# Autodesk Inventor assembly: Ensamblaje
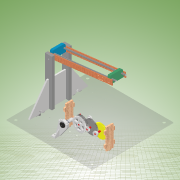
[picture p0: Inventor's stored thumbnail of the model, 180x180]
Saved by Autodesk Inventor 2022 (Build 260153000, 153)
## iProperties
Created: 2022-02-04
Part Number: Ensamblaje
Document SubType Name: Assembly
Designer: Marco
Author: Marco
## Documents named in this file (23)
- C:\Users\steff\Desktop\9noSemestre\Diseño\MiniProyecto\Ensamblaje.iam
- C:\Users\steff\Desktop\9noSemestre\Diseño\MiniProyecto\SoporteDerecha.ipt
- C:\Users\steff\Desktop\9noSemestre\Diseño\MiniProyecto\Varilla.ipt
- C:\Users\steff\Desktop\9noSemestre\Diseño\MiniProyecto\Riel_Lateral_MDF.ipt
- C:\Users\steff\Desktop\9noSemestre\Diseño\MiniProyecto\ColumnaSoporte.ipt
- C:\Users\steff\Desktop\9noSemestre\Diseño\MiniProyecto\SoporteIzquierda.ipt
- C:\Users\steff\Desktop\9noSemestre\Diseño\MiniProyecto\UnionColumnas.ipt
- C:\Users\steff\Desktop\9noSemestre\Diseño\MiniProyecto\SoporteMotor.ipt
- C:\Users\steff\Desktop\9noSemestre\Diseño\MiniProyecto\BaseProyecto.ipt
- C:\Users\steff\Desktop\9noSemestre\Diseño\MiniProyecto\SoporteMotorCierre.ipt
- C:\Users\steff\Desktop\9noSemestre\Diseño\MiniProyecto\dc motor.ipt
- C:\Users\steff\Desktop\9noSemestre\Diseño\MiniProyecto\CaraLateral.ipt
- C:\Users\steff\Desktop\9noSemestre\Diseño\MiniProyecto\Caja_CaraFrontal.ipt
- C:\Users\steff\Desktop\9noSemestre\Diseño\MiniProyecto\AcopleMotor.ipt
- C:\Users\steff\Desktop\9noSemestre\Diseño\MiniProyecto\SoporteEje.ipt
- C:\Users\steff\Desktop\9noSemestre\Diseño\MiniProyecto\Eje.ipt
- C:\Users\steff\Desktop\9noSemestre\Diseño\MiniProyecto\Engranaje.ipt
- C:\Users\steff\Desktop\9noSemestre\Diseño\MiniProyecto\EnsamblajesJuntos.iam
- C:\Users\steff\Desktop\9noSemestre\Diseño\MiniProyecto\libreria\es-ES\AS 1110\AS 1110 - M5 x 16.ipt
- C:\Users\steff\Desktop\9noSemestre\Diseño\MiniProyecto\Transmision_Inf.ipt
- C:\Users\steff\Desktop\9noSemestre\Diseño\MiniProyecto\Transmision_Sup.ipt
- C:\Users\steff\Desktop\9noSemestre\Diseño\MiniProyecto\Engranaje1.ipt
- C:\Users\steff\Desktop\9noSemestre\Diseño\MiniProyecto\Piñon1.ipt
## Components (36 placed, 22 different names)
1. ColumnaSoporte:1 — Coincidencia:1, Coincidencia:3, Coincidencia:6, Coincidencia:8, De rotación:2
2. ColumnaSoporte:2 — Coincidencia:2, Coincidencia:4, Coincidencia:5, Coincidencia:7, De rotación:1
3. UnionColumnas:1 — Coincidencia:3, Coincidencia:4, Coincidencia:5, Coincidencia:6, Coincidencia:21, Coincidencia:31, Coincidencia:92, Coincidencia:93
4. Riel_Lateral_MDF:1 — Coincidencia:7, De rotación:1, Coincidencia:10, Coincidencia:13, Coincidencia:14
5. Riel_Lateral_MDF:2 — Coincidencia:8, De rotación:2, De rotación:3, Coincidencia:9, Coincidencia:11, Coincidencia:12, Coincidencia:90
6. SoporteIzquierda:1 — De rotación:3, Coincidencia:9, Coincidencia:10, Coincidencia:15, Coincidencia:17, Coincidencia:18, Coincidencia:20
7. SoporteDerecha:1 — Coincidencia:11, Coincidencia:12, Coincidencia:13, Coincidencia:14, Coincidencia:16, Coincidencia:19
8. Varilla:1 — Coincidencia:15, Coincidencia:16, Coincidencia:17
9. Varilla:2 — Coincidencia:18, Coincidencia:19, Coincidencia:20
10. AS 1110 - Métrico M5 x 16:1 — Coincidencia:21
11. BaseProyecto:1 — Coincidencia:31, Coincidencia:46, Coincidencia:47, Coincidencia:92, Coincidencia:93, Coincidencia:94, Coincidencia:95
12. SoporteMotor:1 — Coincidencia:32, Coincidencia:33, Coincidencia:34, Coincidencia:35, Coincidencia:47, Coincidencia:48, Coincidencia:49
13. SoporteMotorCierre:1 — Coincidencia:32, Coincidencia:33, Coincidencia:34, Coincidencia:50
14. dc motor:1 — Coincidencia:35, Coincidencia:50, Coincidencia:51, Coincidencia:53
15. CaraLateral:1 — Coincidencia:36, Coincidencia:38, Coincidencia:42, Coincidencia:43, Coincidencia:44, Coincidencia:45, Coincidencia:69, Coincidencia:70, Coincidencia:71, Coincidencia:72, Coincidencia:73, Coincidencia:74
16. CaraLateral:2 — Coincidencia:37, Coincidencia:39, Coincidencia:40, Coincidencia:41, Coincidencia:48, Coincidencia:49, Coincidencia:52, Coincidencia:54, Coincidencia:55, Coincidencia:56, Coincidencia:57, Coincidencia:58, Coincidencia:59, Coincidencia:83, Coincidencia:94, Coincidencia:95
17. Caja_CaraFrontal:1 — Coincidencia:38, Coincidencia:39, Coincidencia:44, Coincidencia:45, Coincidencia:46
18. Caja_CaraFrontal:2 — Coincidencia:36, Coincidencia:37, Coincidencia:40, Coincidencia:41, Coincidencia:42, Coincidencia:43
19. AcopleMotor:1 — Coincidencia:51, Coincidencia:52, Coincidencia:53, Coincidencia:96, Coincidencia:97, Coincidencia:98
20. SoporteEje:1 — Coincidencia:54, Coincidencia:55, Coincidencia:60, Coincidencia:61, Coincidencia:65
21. SoporteEje:2 — Coincidencia:56, Coincidencia:57, Coincidencia:62, Coincidencia:63, Coincidencia:64, Coincidencia:76
22. SoporteEje:3 — Coincidencia:58, Coincidencia:59, Coincidencia:66, Coincidencia:67, Coincidencia:68, Coincidencia:75
23. Eje:1 — Coincidencia:60, Coincidencia:61, Coincidencia:65, Coincidencia:79, Coincidencia:80, Coincidencia:99, Coincidencia:100
24. Eje:2 — Coincidencia:62, Coincidencia:63, Coincidencia:64, Coincidencia:76, Coincidencia:81, Coincidencia:82, Coincidencia:101, Coincidencia:102
25. Eje:3 — Coincidencia:66, Coincidencia:67, Coincidencia:68, Coincidencia:75, Coincidencia:77, Coincidencia:78
26. SoporteEje:4 — Coincidencia:69, Coincidencia:70
27. SoporteEje:5 — Coincidencia:71, Coincidencia:74
28. SoporteEje:6 — Coincidencia:72, Coincidencia:73, Coincidencia:86, Coincidencia:88, Coincidencia:89
29. Engranaje:1 — Coincidencia:77, Coincidencia:78, Coincidencia:85
30. EnsamblajesJuntos:1 [sub-assembly] — Coincidencia:79, Coincidencia:80, Coincidencia:83, Coincidencia:84
31. EnsamblajesJuntos:2 [sub-assembly] — Coincidencia:81, Coincidencia:82, Coincidencia:84, Coincidencia:85
32. Transmision_Inf:1 — Coincidencia:86, Cilíndrica:1, Coincidencia:87, Coincidencia:88, Coincidencia:89
33. Transmision_Sup:1 — Cilíndrica:1, Coincidencia:87, Coincidencia:90
34. Eje:4 — Coincidencia:96, Coincidencia:97, Coincidencia:98
35. Engranaje1:1 — Coincidencia:99, Coincidencia:100
36. Piñon1:1 — Coincidencia:101, Coincidencia:102
## Relationships (96: Mate 92, RevoluteJoint 3, CylindricalJoint 1)
- Coincidencia:1 [Mate]: ColumnaSoporte:1
- Coincidencia:2 [Mate]: ColumnaSoporte:2
- Coincidencia:3 [Mate]: ColumnaSoporte:1 ↔ UnionColumnas:1
- Coincidencia:4 [Mate]: ColumnaSoporte:2 ↔ UnionColumnas:1
- Coincidencia:5 [Mate]: ColumnaSoporte:2 ↔ UnionColumnas:1
- Coincidencia:6 [Mate]: ColumnaSoporte:1 ↔ UnionColumnas:1
- Coincidencia:7 [Mate]: ColumnaSoporte:2 ↔ Riel_Lateral_MDF:1
- Coincidencia:8 [Mate]: ColumnaSoporte:1 ↔ Riel_Lateral_MDF:2
- De rotación:1 [RevoluteJoint]: ColumnaSoporte:2 ↔ Riel_Lateral_MDF:1
- De rotación:2 [RevoluteJoint]: ColumnaSoporte:1 ↔ Riel_Lateral_MDF:2
- De rotación:3 [RevoluteJoint]: Riel_Lateral_MDF:2 ↔ SoporteIzquierda:1
- Coincidencia:9 [Mate]: Riel_Lateral_MDF:2 ↔ SoporteIzquierda:1
- Coincidencia:10 [Mate]: Riel_Lateral_MDF:1 ↔ SoporteIzquierda:1
- Coincidencia:11 [Mate]: Riel_Lateral_MDF:2 ↔ SoporteDerecha:1
- Coincidencia:12 [Mate]: Riel_Lateral_MDF:2 ↔ SoporteDerecha:1
- Coincidencia:13 [Mate]: Riel_Lateral_MDF:1 ↔ SoporteDerecha:1
- Coincidencia:14 [Mate]: Riel_Lateral_MDF:1 ↔ SoporteDerecha:1
- Coincidencia:15 [Mate]: SoporteIzquierda:1 ↔ Varilla:1
- Coincidencia:16 [Mate]: SoporteDerecha:1 ↔ Varilla:1
- Coincidencia:17 [Mate]: SoporteIzquierda:1 ↔ Varilla:1
- Coincidencia:18 [Mate]: SoporteIzquierda:1 ↔ Varilla:2
- Coincidencia:19 [Mate]: SoporteDerecha:1 ↔ Varilla:2
- Coincidencia:20 [Mate]: SoporteIzquierda:1 ↔ Varilla:2
- Coincidencia:21 [Mate]: UnionColumnas:1 ↔ AS 1110 - Métrico M5 x 16:1
- Coincidencia:31 [Mate]: UnionColumnas:1 ↔ BaseProyecto:1
- Coincidencia:32 [Mate]: SoporteMotor:1 ↔ SoporteMotorCierre:1
- Coincidencia:33 [Mate]: SoporteMotor:1 ↔ SoporteMotorCierre:1
- Coincidencia:34 [Mate]: SoporteMotor:1 ↔ SoporteMotorCierre:1
- Coincidencia:35 [Mate]: SoporteMotor:1 ↔ dc motor:1
- Coincidencia:36 [Mate]: CaraLateral:1 ↔ Caja_CaraFrontal:2
- Coincidencia:37 [Mate]: CaraLateral:2 ↔ Caja_CaraFrontal:2
- Coincidencia:38 [Mate]: CaraLateral:1 ↔ Caja_CaraFrontal:1
- Coincidencia:39 [Mate]: CaraLateral:2 ↔ Caja_CaraFrontal:1
- Coincidencia:40 [Mate]: CaraLateral:2 ↔ Caja_CaraFrontal:2
- Coincidencia:41 [Mate]: CaraLateral:2 ↔ Caja_CaraFrontal:2
- Coincidencia:42 [Mate]: CaraLateral:1 ↔ Caja_CaraFrontal:2
- Coincidencia:43 [Mate]: CaraLateral:1 ↔ Caja_CaraFrontal:2
- Coincidencia:44 [Mate]: CaraLateral:1 ↔ Caja_CaraFrontal:1
- Coincidencia:45 [Mate]: CaraLateral:1 ↔ Caja_CaraFrontal:1
- Coincidencia:46 [Mate]: BaseProyecto:1 ↔ Caja_CaraFrontal:1
- Coincidencia:47 [Mate]: BaseProyecto:1 ↔ SoporteMotor:1
- Coincidencia:48 [Mate] (28 mm): SoporteMotor:1 ↔ CaraLateral:2
- Coincidencia:49 [Mate]: SoporteMotor:1 ↔ CaraLateral:2
- Coincidencia:50 [Mate]: SoporteMotorCierre:1 ↔ dc motor:1
- Coincidencia:51 [Mate]: dc motor:1 ↔ AcopleMotor:1
- Coincidencia:52 [Mate]: CaraLateral:2 ↔ AcopleMotor:1
- Coincidencia:53 [Mate]: dc motor:1 ↔ AcopleMotor:1
- Coincidencia:54 [Mate]: CaraLateral:2 ↔ SoporteEje:1
- Coincidencia:55 [Mate]: CaraLateral:2 ↔ SoporteEje:1
- Coincidencia:56 [Mate]: CaraLateral:2 ↔ SoporteEje:2
- Coincidencia:57 [Mate]: CaraLateral:2 ↔ SoporteEje:2
- Coincidencia:58 [Mate]: CaraLateral:2 ↔ SoporteEje:3
- Coincidencia:59 [Mate]: CaraLateral:2 ↔ SoporteEje:3
- Coincidencia:60 [Mate]: SoporteEje:1 ↔ Eje:1
- Coincidencia:61 [Mate]: SoporteEje:1 ↔ Eje:1
- Coincidencia:62 [Mate]: SoporteEje:2 ↔ Eje:2
- Coincidencia:63 [Mate]: SoporteEje:2 ↔ Eje:2
- Coincidencia:64 [Mate]: SoporteEje:2 ↔ Eje:2
- Coincidencia:65 [Mate]: SoporteEje:1 ↔ Eje:1
- Coincidencia:66 [Mate]: SoporteEje:3 ↔ Eje:3
- Coincidencia:67 [Mate]: SoporteEje:3 ↔ Eje:3
- Coincidencia:68 [Mate]: SoporteEje:3 ↔ Eje:3
- Coincidencia:69 [Mate]: CaraLateral:1 ↔ SoporteEje:4
- Coincidencia:70 [Mate]: CaraLateral:1 ↔ SoporteEje:4
- Coincidencia:71 [Mate]: CaraLateral:1 ↔ SoporteEje:5
- Coincidencia:72 [Mate]: CaraLateral:1 ↔ SoporteEje:6
- Coincidencia:73 [Mate]: CaraLateral:1 ↔ SoporteEje:6
- Coincidencia:74 [Mate]: CaraLateral:1 ↔ SoporteEje:5
- Coincidencia:75 [Mate]: SoporteEje:3 ↔ Eje:3
- Coincidencia:76 [Mate]: SoporteEje:2 ↔ Eje:2
- Coincidencia:77 [Mate]: Eje:3 ↔ Engranaje:1
- Coincidencia:78 [Mate]: Eje:3 ↔ Engranaje:1
- Coincidencia:79 [Mate]: Eje:1 ↔ EnsamblajesJuntos:1
- Coincidencia:80 [Mate]: Eje:1 ↔ EnsamblajesJuntos:1
- Coincidencia:81 [Mate]: Eje:2 ↔ EnsamblajesJuntos:2
- Coincidencia:82 [Mate]: Eje:2 ↔ EnsamblajesJuntos:2
- Coincidencia:83 [Mate]: CaraLateral:2 ↔ EnsamblajesJuntos:1
- Coincidencia:84 [Mate]: EnsamblajesJuntos:1 ↔ EnsamblajesJuntos:2
- Coincidencia:85 [Mate]: Engranaje:1 ↔ EnsamblajesJuntos:2
- Coincidencia:86 [Mate]: SoporteEje:6 ↔ Transmision_Inf:1
- Cilíndrica:1 [CylindricalJoint]: Transmision_Inf:1 ↔ Transmision_Sup:1
- Coincidencia:87 [Mate]: Transmision_Inf:1 ↔ Transmision_Sup:1
- Coincidencia:88 [Mate]: SoporteEje:6 ↔ Transmision_Inf:1
- Coincidencia:89 [Mate]: SoporteEje:6 ↔ Transmision_Inf:1
- Coincidencia:90 [Mate]: Riel_Lateral_MDF:2 ↔ Transmision_Sup:1
- Coincidencia:92 [Mate]: UnionColumnas:1 ↔ BaseProyecto:1
- Coincidencia:93 [Mate]: UnionColumnas:1 ↔ BaseProyecto:1
- Coincidencia:94 [Mate]: BaseProyecto:1 ↔ CaraLateral:2
- Coincidencia:95 [Mate]: BaseProyecto:1 ↔ CaraLateral:2
- Coincidencia:96 [Mate]: AcopleMotor:1 ↔ Eje:4
- Coincidencia:97 [Mate]: AcopleMotor:1 ↔ Eje:4
- Coincidencia:98 [Mate]: AcopleMotor:1 ↔ Eje:4
- Coincidencia:99 [Mate]: Eje:1 ↔ Engranaje1:1
- Coincidencia:100 [Mate]: Eje:1 ↔ Engranaje1:1
- Coincidencia:101 [Mate]: Eje:2 ↔ Piñon1:1
- Coincidencia:102 [Mate]: Eje:2 ↔ Piñon1:1
